# Autodesk Inventor assembly: Claw2017-18
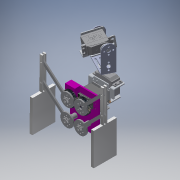
[picture p0: Inventor's stored thumbnail of the model, 180x180]
Saved by Autodesk Inventor 2017 (Build 210142000, 142)
## iProperties
Created: 2017-09-28
Part Number: Claw2017-18
Document SubType Name: Assembly
Designer: User
Author: User
## Documents named in this file (11)
- C:\Robotics\CAD\2017-18_CAD\Claw2017-18.iam
- C:\Robotics\CAD\2017-18_CAD\ClawServoHolder.ipt
- C:\Robotics\CAD\COTSParts\Tetrix\Tetrix servo 180.ipt
- C:\Robotics\CAD\COTSParts\Tetrix\Tetrix Gear 40T.ipt
- C:\Robotics\CAD\2017-18_CAD\ClawLinkage.ipt
- C:\Robotics\CAD\2017-18_CAD\2BarClawPaddle.ipt
- C:\Robotics\CAD\COTSParts\Vex\91259A576_ALLOY STEEL SHOULDER SCREW.ipt
- C:\Robotics\CAD\COTSParts\Vex\91259A581_ALLOY STEEL SHOULDER SCREW.ipt
- C:\Robotics\CAD\2017-18_CAD\ClawSpacer.ipt
- C:\Robotics\CAD\COTSParts\Tetrix\Tetrix bracket - single servo.ipt
- C:\Robotics\CAD\2017-18_CAD\TheClaw.iam
## Components (17 placed, 10 different names)
1. ClawServoHolder:1 — Mate:5, Mate:6, Mate:7, Mate:11, Mate:12, Mate:43, Mate:44, Mate:45, Mate:46, Mate:53, Mate:54, Mate:55
2. Tetrix servo 180:1 — Mate:5, Mate:6, Mate:7, Mate:9, Mate:10, Mate:56, Mate:57
3. Tetrix Gear 40T:1 — Mate:9, Mate:10, Flush:5, Mate:19, Mate:20, Mate:21
4. Tetrix Gear 40T:2 — Mate:11, Mate:12, Flush:5, Mate:22, Mate:23, Mate:24
5. ClawLinkage:1 — Mate:19, Mate:20, Mate:21, Insert:1
6. ClawLinkage:2 — Mate:22, Mate:23, Mate:24, Mate:42
7. 2BarClawPaddle:2 — Mate:42, Insert:2
8. 2BarClawPaddle:3 — Insert:1, Insert:3
9. 91259A576_ALLOY STEEL SHOULDER SCREW:1 — Mate:43, Mate:44, Flush:6, Flush:7
10. 91259A581_ALLOY STEEL SHOULDER SCREW:3 — Mate:45, Flush:6, Mate:47, Mate:48, Mate:52
11. 91259A581_ALLOY STEEL SHOULDER SCREW:4 — Mate:46, Flush:7, Mate:49, Mate:50, Mate:51
12. ClawLinkage:3 — Mate:47, Mate:48, Insert:3
13. ClawLinkage:4 — Mate:49, Mate:50, Insert:2
14. ClawSpacer:1 — Mate:51, Mate:53
15. ClawSpacer:2 — Mate:52, Mate:54
16. Tetrix bracket - single servo:1 — Mate:55, Mate:56, Insert:4, Insert:5, Mate:57
17. TheClaw:1 [sub-assembly] — Insert:4, Insert:5
## Relationships (37: Mate 29, Insert 5, Flush 3)
- Mate:5: ClawServoHolder:1 ↔ Tetrix servo 180:1
- Mate:6: ClawServoHolder:1 ↔ Tetrix servo 180:1
- Mate:7: ClawServoHolder:1 ↔ Tetrix servo 180:1
- Mate:9: Tetrix servo 180:1 ↔ Tetrix Gear 40T:1
- Mate:10: Tetrix servo 180:1 ↔ Tetrix Gear 40T:1
- Mate:11: ClawServoHolder:1 ↔ Tetrix Gear 40T:2
- Mate:12: ClawServoHolder:1 ↔ Tetrix Gear 40T:2
- Flush:5: Tetrix Gear 40T:1 ↔ Tetrix Gear 40T:2
- Mate:19: Tetrix Gear 40T:1 ↔ ClawLinkage:1
- Mate:20: Tetrix Gear 40T:1 ↔ ClawLinkage:1
- Mate:21: Tetrix Gear 40T:1 ↔ ClawLinkage:1
- Mate:22: Tetrix Gear 40T:2 ↔ ClawLinkage:2
- Mate:23: Tetrix Gear 40T:2 ↔ ClawLinkage:2
- Mate:24: Tetrix Gear 40T:2 ↔ ClawLinkage:2
- Insert:1: ClawLinkage:1 ↔ 2BarClawPaddle:3
- Mate:42: ClawLinkage:2 ↔ 2BarClawPaddle:2
- Mate:43: ClawServoHolder:1 ↔ 91259A576_ALLOY STEEL SHOULDER SCREW:1
- Mate:44: ClawServoHolder:1 ↔ 91259A576_ALLOY STEEL SHOULDER SCREW:1
- Mate:45: ClawServoHolder:1 ↔ 91259A581_ALLOY STEEL SHOULDER SCREW:3
- Flush:6: 91259A576_ALLOY STEEL SHOULDER SCREW:1 ↔ 91259A581_ALLOY STEEL SHOULDER SCREW:3
- Mate:46: ClawServoHolder:1 ↔ 91259A581_ALLOY STEEL SHOULDER SCREW:4
- Flush:7: 91259A576_ALLOY STEEL SHOULDER SCREW:1 ↔ 91259A581_ALLOY STEEL SHOULDER SCREW:4
- Mate:47: 91259A581_ALLOY STEEL SHOULDER SCREW:3 ↔ ClawLinkage:3
- Mate:48: 91259A581_ALLOY STEEL SHOULDER SCREW:3 ↔ ClawLinkage:3
- Mate:49: 91259A581_ALLOY STEEL SHOULDER SCREW:4 ↔ ClawLinkage:4
- Mate:50: 91259A581_ALLOY STEEL SHOULDER SCREW:4 ↔ ClawLinkage:4
- Insert:2: 2BarClawPaddle:2 ↔ ClawLinkage:4
- Insert:3: 2BarClawPaddle:3 ↔ ClawLinkage:3
- Mate:51: 91259A581_ALLOY STEEL SHOULDER SCREW:4 ↔ ClawSpacer:1
- Mate:52: 91259A581_ALLOY STEEL SHOULDER SCREW:3 ↔ ClawSpacer:2
- Mate:53: ClawServoHolder:1 ↔ ClawSpacer:1
- Mate:54: ClawServoHolder:1 ↔ ClawSpacer:2
- Mate:55 (2.54 mm): ClawServoHolder:1 ↔ Tetrix bracket - single servo:1
- Mate:56: Tetrix servo 180:1 ↔ Tetrix bracket - single servo:1
- Insert:4: Tetrix bracket - single servo:1 ↔ TheClaw:1
- Insert:5: Tetrix bracket - single servo:1 ↔ TheClaw:1
- Mate:57: Tetrix servo 180:1 ↔ Tetrix bracket - single servo:1
